# Autodesk Inventor assembly: HalfLeftTest
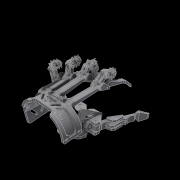
[picture p0: Inventor's stored thumbnail of the model, 180x180]
Saved by Autodesk Inventor 2015 (Build 190159000, 159)
## iProperties
Created: 2014-10-25
Part Number: HalfLeftTest
Document SubType Name: Assembly
Designer: Val
Mass: 54.0122 g
Surface Area: 465.408 cm^2
Volume: 54.0122 cm^3
Density: 1 g/cm^3
Author: Val
## Documents named in this file (31)
- F:\Exo\Models\3D\HandLeft.iam
- F:\Exo\Models\3D\HandShockPlateLeft.ipt
- F:\Exo\Models\3D\VibroKnuckle.ipt
- F:\Exo\Models\3D\KnuckleSide.ipt
- F:\Exo\Models\3D\ThumbShockPlateLeft.ipt
- F:\Exo\Models\3D\ThumbMount.ipt
- F:\Exo\Models\3D\MetacarpusIndex.ipt
- F:\Exo\Models\3D\MetacarpusMiddle.ipt
- F:\Exo\Models\3D\MetacarpusRing.ipt
- F:\Exo\Models\3D\MetacarpusPinky.ipt
- F:\Exo\Models\3D\MetacarpusThumb.ipt
- F:\Exo\Models\3D\ProxPhalangeIndex.ipt
- F:\Exo\Models\3D\ProxPhalangeMiddle.ipt
- F:\Exo\Models\3D\ProxPhalangeRing.ipt
- F:\Exo\Models\3D\ProxPhalangePinky.ipt
- F:\Exo\Models\3D\DistPhalangeIndex.ipt
- F:\Exo\Models\3D\DistPhalangeMiddle.ipt
- F:\Exo\Models\3D\DistPhalangeRing.ipt
- F:\Exo\Models\3D\DistPhalangePinky.ipt
- F:\Exo\Models\3D\DistPhalangeThumb.ipt
- F:\Exo\Models\3D\HandRibLeft.ipt
- F:\Exo\Models\3D\IndexRouter.ipt
- F:\Exo\Models\3D\MiddleRouter.ipt
- F:\Exo\Models\3D\RingRouter.ipt
- F:\Exo\Models\3D\PinkyRouter.ipt
- F:\Exo\Models\3D\ThumbRouter.ipt
- F:\Exo\Models\3D\VibroMount.ipt
- F:\Exo\Models\3D\ChainLink.ipt
- F:\Exo\Models\3D\ChainTooth.ipt
- F:\Exo\Models\3D\ChainGear.ipt
- F:\Exo\Models\3D\ProxPhalangeThumb.ipt
## Components (167 placed, 30 different names)
1. HandShockPlateLeft:1 — Mate:72, Mate:73, Mate:78, Mate:79, Mate:80, Mate:81, Mate:137, Mate:139
2. ThumbShockPlateLeft:1 — Mate:72, Mate:73, Mate:74, Mate:75
3. ThumbMount:1 — Mate:74, Mate:75, Mate:76, Mate:77
4. VibroKnuckle:1 — Mate:82, Mate:83, Mate:94, Mate:95, Mate:410, Mate:411, Mate:413
5. VibroKnuckle:2 — Mate:84, Mate:85, Mate:96, Mate:97, Mate:347, Mate:348, Mate:349, Mate:350
6. VibroKnuckle:3 — Mate:86, Mate:87, Mate:98, Mate:99, Mate:142, Mate:143, Mate:144, Mate:145
7. VibroKnuckle:4 — Mate:88, Mate:89, Mate:286, Mate:287
8. VibroKnuckle:5 — Mate:90, Mate:91, Mate:100, Mate:101, Mate:283, Mate:284, Mate:285
9. KnuckleSide:1 — Mate:102, Mate:104
10. KnuckleSide:2 — Mate:105, Mate:107
11. KnuckleSide:3 — Mate:108, Mate:109, Mate:110
12. KnuckleSide:4 — Mate:111, Mate:112, Mate:113
13. KnuckleSide:5 — Mate:114, Mate:115, Mate:116
14. KnuckleSide:6 — Mate:117, Mate:118, Mate:119
15. KnuckleSide:7 — Mate:120, Mate:121, Mate:122
16. KnuckleSide:8 — Mate:123, Mate:124, Mate:125
17. KnuckleSide:9 — Mate:129, Mate:130, Mate:131
18. KnuckleSide:10 — Mate:126, Mate:127, Mate:128
19. MetacarpusIndex:1 — Mate:78, Mate:82, Mate:83, Mate:108, Mate:110, Mate:111, Mate:113
20. MetacarpusMiddle:2 — Mate:79, Mate:84, Mate:85, Mate:114, Mate:116, Mate:117, Mate:119
21. MetacarpusRing:3 — Mate:80, Mate:86, Mate:87, Mate:120, Mate:122, Mate:123, Mate:125
22. MetacarpusPinky:4 — Mate:81, Mate:90, Mate:91, Mate:126, Mate:128, Mate:129, Mate:131
23. MetacarpusThumb:5 — Mate:76, Mate:77, Mate:88, Mate:89, Mate:102, Mate:104, Mate:105, Mate:107
24. ProxPhalangeIndex:1 — Mate:94, Mate:95, Mate:109, Mate:112, Mate:135
25. ProxPhalangeMiddle:2 — Mate:96, Mate:97, Mate:115, Mate:118, Mate:134
26. ProxPhalangeRing:3 — Mate:98, Mate:99, Mate:121, Mate:124, Mate:133
27. ProxPhalangePinky:4 — Mate:100, Mate:101, Mate:127, Mate:130, Mate:132
28. DistPhalangeIndex:1 — Mate:135
29. DistPhalangeMiddle:1 — Mate:134
30. DistPhalangeRing:1 — Mate:133
31. DistPhalangePinky:1 — Mate:132
32. DistPhalangeThumb:1
33. HandRibLeft:1 — Mate:137, Mate:139
34. IndexRouter:1
35. MiddleRouter:1
36. RingRouter:1
37. PinkyRouter:1
38. ThumbRouter:1
39. VibroMount:1 — Mate:142, Mate:143, Mate:148, Mate:180
40. VibroMount:2 — Mate:144, Mate:145, Mate:148, Mate:179
41. ChainLink:1 — Mate:149, Mate:150, Mate:181
42. ChainTooth:1 — Mate:149, Mate:150, Mate:151, Mate:152, Mate:154, Mate:155, Mate:156, Flush:4, Flush:15
43. ChainLink:2 — Mate:156, Flush:1, Mate:181, Mate:216
44. ChainLink:3 — Mate:154, Mate:155, Flush:1, Mate:178
45. ChainLink:4 — Mate:151, Mate:152, Mate:171
46. ChainLink:7 — Mate:172
47. ChainTooth:2 — Flush:5, Flush:6
48. ChainLink:8 — Mate:173
49. ChainLink:9 — Mate:176
50. ChainLink:10 — Mate:174
51. ChainLink:11 — Mate:175
52. ChainTooth:3 — Flush:7
53. ChainLink:12 — Mate:177
54. ChainLink:13 — Mate:182
55. ChainLink:14 — Mate:182, Mate:222, Mate:223
56. ChainTooth:4 — Mate:171, Flush:4, Flush:5, Mate:172, Mate:173, Mate:178
57. ChainTooth:5 — Flush:6, Mate:174, Flush:7, Mate:175, Mate:176, Mate:177
58. VibroKnuckle:6 — Mate:179, Mate:180, Mate:218, Mate:219, Mate:220, Mate:221
59. ChainTooth:7 — Mate:223
60. ChainLink:21
61. ChainLink:22
62. ChainLink:23
63. ChainTooth:8
64. ChainLink:24
65. ChainLink:25 — Mate:215
66. ChainLink:26 — Mate:214
67. ChainTooth:10
68. ChainTooth:11 — Mate:214, Mate:215, Mate:216, Flush:15
69. ChainGear:1 — Mate:218, Mate:220, Mate:222
70. ChainGear:2 — Mate:219, Mate:221
71. VibroMount:3 — Mate:285
72. VibroMount:4 — Mate:283, Mate:284
73. ChainLink:27 — Flush:36, Flush:37
74. ChainTooth:12
75. ChainLink:28
76. ChainLink:29
77. ChainLink:30 — Flush:28, Flush:29, Flush:37
78. ChainLink:31 — Flush:29, Flush:30
79. ChainTooth:13
80. ChainLink:32
81. ChainLink:33
82. ChainLink:34 — Flush:30, Flush:31
83. ChainLink:35 — Flush:27, Flush:31, Flush:32
84. ChainTooth:14
85. ChainLink:36
86. ChainLink:37
87. ChainLink:38 — Flush:32, Flush:33
88. ChainTooth:15
89. ChainTooth:16
90. VibroKnuckle:7
91. ChainTooth:17
92. ChainLink:39
93. ChainLink:40 — Flush:33, Flush:34
94. ChainLink:41 — Flush:34, Flush:35
95. ChainTooth:18
96. ChainLink:42
97. ChainLink:43
98. ChainLink:44 — Flush:35, Flush:36
99. ChainTooth:19
100. ChainTooth:20
101. ChainGear:3 — Flush:27
102. ChainGear:4 — Flush:28
103. ProxPhalangeThumb:1 — Mate:286, Mate:287
104. VibroMount:5 — Mate:347, Mate:348
105. VibroMount:6 — Mate:349, Mate:350
106. ChainLink:45
107. ChainTooth:21
108. ChainLink:46
109. ChainLink:47
110. ChainLink:48
111. ChainLink:49
112. ChainTooth:22
113. ChainLink:50
114. ChainLink:51
115. ChainLink:52
116. ChainLink:53
117. ChainTooth:23
118. ChainLink:54
119. ChainLink:55
120. ChainLink:56
121. ChainTooth:24
122. ChainTooth:25
123. VibroKnuckle:8
124. ChainTooth:26
125. ChainLink:57
126. ChainLink:58
127. ChainLink:59
128. ChainTooth:27
129. ChainLink:60
130. ChainLink:61
131. ChainLink:62
132. ChainTooth:28
133. ChainTooth:29
134. ChainGear:5
135. ChainGear:6
136. VibroMount:7 — Mate:410, Mate:411, Mate:412
137. VibroMount:8 — Mate:413
138. ChainLink:63
139. ChainTooth:30
140. ChainLink:64
141. ChainLink:65
142. ChainLink:66
143. ChainLink:67
144. ChainTooth:31
145. ChainLink:68
146. ChainLink:69
147. ChainLink:70
148. ChainLink:71
149. ChainTooth:32
150. ChainLink:72
151. ChainLink:73
152. ChainLink:74
153. ChainTooth:33
154. ChainTooth:34
155. VibroKnuckle:9 — Mate:412
156. ChainTooth:35
157. ChainLink:75
158. ChainLink:76
159. ChainLink:77
160. ChainTooth:36
161. ChainLink:78
162. ChainLink:79
163. ChainLink:80
164. ChainTooth:37
165. ChainTooth:38
166. ChainGear:7
167. ChainGear:8
## Relationships (392: Mate 315, Flush 77)
- Mate:72: HandShockPlateLeft:1 ↔ ThumbShockPlateLeft:1
- Mate:73: HandShockPlateLeft:1 ↔ ThumbShockPlateLeft:1
- Mate:74: ThumbShockPlateLeft:1 ↔ ThumbMount:1
- Mate:75: ThumbShockPlateLeft:1 ↔ ThumbMount:1
- Mate:76: ThumbMount:1 ↔ MetacarpusThumb:5
- Mate:77: ThumbMount:1 ↔ MetacarpusThumb:5
- Mate:78: HandShockPlateLeft:1 ↔ MetacarpusIndex:1
- Mate:79: HandShockPlateLeft:1 ↔ MetacarpusMiddle:2
- Mate:80: HandShockPlateLeft:1 ↔ MetacarpusRing:3
- Mate:81: HandShockPlateLeft:1 ↔ MetacarpusPinky:4
- Mate:82: VibroKnuckle:1 ↔ MetacarpusIndex:1
- Mate:83: VibroKnuckle:1 ↔ MetacarpusIndex:1
- Mate:84: VibroKnuckle:2 ↔ MetacarpusMiddle:2
- Mate:85: VibroKnuckle:2 ↔ MetacarpusMiddle:2
- Mate:86: VibroKnuckle:3 ↔ MetacarpusRing:3
- Mate:87: VibroKnuckle:3 ↔ MetacarpusRing:3
- Mate:88: VibroKnuckle:4 ↔ MetacarpusThumb:5
- Mate:89: VibroKnuckle:4 ↔ MetacarpusThumb:5
- Mate:90: VibroKnuckle:5 ↔ MetacarpusPinky:4
- Mate:91: VibroKnuckle:5 ↔ MetacarpusPinky:4
- Mate:94: VibroKnuckle:1 ↔ ProxPhalangeIndex:1
- Mate:95: VibroKnuckle:1 ↔ ProxPhalangeIndex:1
- Mate:96: VibroKnuckle:2 ↔ ProxPhalangeMiddle:2
- Mate:97: VibroKnuckle:2 ↔ ProxPhalangeMiddle:2
- Mate:98: VibroKnuckle:3 ↔ ProxPhalangeRing:3
- Mate:99: VibroKnuckle:3 ↔ ProxPhalangeRing:3
- Mate:100: VibroKnuckle:5 ↔ ProxPhalangePinky:4
- Mate:101: VibroKnuckle:5 ↔ ProxPhalangePinky:4
- Mate:102: KnuckleSide:1 ↔ MetacarpusThumb:5
- Mate:104: KnuckleSide:1 ↔ MetacarpusThumb:5
- Mate:105: KnuckleSide:2 ↔ MetacarpusThumb:5
- Mate:107: KnuckleSide:2 ↔ MetacarpusThumb:5
- Mate:108: KnuckleSide:3 ↔ MetacarpusIndex:1
- Mate:109: KnuckleSide:3 ↔ ProxPhalangeIndex:1
- Mate:110: KnuckleSide:3 ↔ MetacarpusIndex:1
- Mate:111: KnuckleSide:4 ↔ MetacarpusIndex:1
- Mate:112: KnuckleSide:4 ↔ ProxPhalangeIndex:1
- Mate:113: KnuckleSide:4 ↔ MetacarpusIndex:1
- Mate:114: KnuckleSide:5 ↔ MetacarpusMiddle:2
- Mate:115: KnuckleSide:5 ↔ ProxPhalangeMiddle:2
- Mate:116: KnuckleSide:5 ↔ MetacarpusMiddle:2
- Mate:117: KnuckleSide:6 ↔ MetacarpusMiddle:2
- Mate:118: KnuckleSide:6 ↔ ProxPhalangeMiddle:2
- Mate:119: KnuckleSide:6 ↔ MetacarpusMiddle:2
- Mate:120: KnuckleSide:7 ↔ MetacarpusRing:3
- Mate:121: KnuckleSide:7 ↔ ProxPhalangeRing:3
- Mate:122: KnuckleSide:7 ↔ MetacarpusRing:3
- Mate:123: KnuckleSide:8 ↔ MetacarpusRing:3
- Mate:124: KnuckleSide:8 ↔ ProxPhalangeRing:3
- Mate:125: KnuckleSide:8 ↔ MetacarpusRing:3
- Mate:126: KnuckleSide:10 ↔ MetacarpusPinky:4
- Mate:127: KnuckleSide:10 ↔ ProxPhalangePinky:4
- Mate:128: KnuckleSide:10 ↔ MetacarpusPinky:4
- Mate:129: KnuckleSide:9 ↔ MetacarpusPinky:4
- Mate:130: KnuckleSide:9 ↔ ProxPhalangePinky:4
- Mate:131: KnuckleSide:9 ↔ MetacarpusPinky:4
- Mate:132: ProxPhalangePinky:4 ↔ DistPhalangePinky:1
- Mate:133: ProxPhalangeRing:3 ↔ DistPhalangeRing:1
- Mate:134: ProxPhalangeMiddle:2 ↔ DistPhalangeMiddle:1
- Mate:135: ProxPhalangeIndex:1 ↔ DistPhalangeIndex:1
- Mate:137: HandShockPlateLeft:1 ↔ HandRibLeft:1
- Mate:139: HandShockPlateLeft:1 ↔ HandRibLeft:1
- Mate:142: VibroKnuckle:3 ↔ VibroMount:1
- Mate:143: VibroKnuckle:3 ↔ VibroMount:1
- Mate:144: VibroKnuckle:3 ↔ VibroMount:2
- Mate:145: VibroKnuckle:3 ↔ VibroMount:2
- Mate:148: VibroMount:1 ↔ VibroMount:2
- Mate:149: ChainLink:1 ↔ ChainTooth:1
- Mate:150: ChainLink:1 ↔ ChainTooth:1
- Mate:151: ChainTooth:1 ↔ ChainLink:4
- Mate:152: ChainTooth:1 ↔ ChainLink:4
- Mate:154: ChainTooth:1 ↔ ChainLink:3
- Mate:155: ChainTooth:1 ↔ ChainLink:3
- Mate:156: ChainTooth:1 ↔ ChainLink:2
- Flush:1: ChainLink:2 ↔ ChainLink:3
- [Mate]: ChainLink:7 ↔ ChainTooth:2
- [Mate]: ChainLink:7 ↔ ChainTooth:2
- [Mate]: ChainTooth:2 ↔ ChainLink:10
- [Mate]: ChainTooth:2 ↔ ChainLink:10
- [Mate]: ChainTooth:2 ↔ ChainLink:9
- [Mate]: ChainTooth:2 ↔ ChainLink:9
- [Mate]: ChainTooth:2 ↔ ChainLink:8
- [Flush]: ChainLink:8 ↔ ChainLink:9
- [Mate]: ChainLink:11 ↔ ChainTooth:3
- [Mate]: ChainLink:11 ↔ ChainTooth:3
- [Mate]: ChainTooth:3 ↔ ChainLink:14
- [Mate]: ChainTooth:3 ↔ ChainLink:14
- [Mate]: ChainTooth:3 ↔ ChainLink:13
- [Mate]: ChainTooth:3 ↔ ChainLink:13
- [Mate]: ChainTooth:3 ↔ ChainLink:12
- [Flush]: ChainLink:12 ↔ ChainLink:13
- Mate:171: ChainLink:4 ↔ ChainTooth:4
- Flush:4: ChainTooth:1 ↔ ChainTooth:4
- Flush:5: ChainTooth:2 ↔ ChainTooth:4
- Mate:172: ChainLink:7 ↔ ChainTooth:4
- Mate:173: ChainLink:8 ↔ ChainTooth:4
- Flush:6: ChainTooth:2 ↔ ChainTooth:5
- Mate:174: ChainLink:10 ↔ ChainTooth:5
- Flush:7: ChainTooth:3 ↔ ChainTooth:5
- Mate:175: ChainLink:11 ↔ ChainTooth:5
- Mate:176: ChainLink:9 ↔ ChainTooth:5
- Mate:177: ChainLink:12 ↔ ChainTooth:5
- Mate:178: ChainLink:3 ↔ ChainTooth:4
- Mate:179: VibroMount:2 ↔ VibroKnuckle:6
- Mate:180: VibroMount:1 ↔ VibroKnuckle:6
- Mate:181: ChainLink:1 ↔ ChainLink:2
- Mate:182: ChainLink:13 ↔ ChainLink:14
- [Mate]: ChainTooth:7 ↔ ChainLink:22
- [Mate]: ChainTooth:7 ↔ ChainLink:22
- [Mate]: ChainTooth:7 ↔ ChainLink:21
- [Mate]: ChainTooth:7 ↔ ChainLink:21
- [Mate]: ChainLink:23 ↔ ChainTooth:8
- [Mate]: ChainLink:23 ↔ ChainTooth:8
- [Mate]: ChainTooth:8 ↔ ChainLink:26
- [Mate]: ChainTooth:8 ↔ ChainLink:26
- [Mate]: ChainTooth:8 ↔ ChainLink:25
- [Mate]: ChainTooth:8 ↔ ChainLink:25
- [Mate]: ChainTooth:8 ↔ ChainLink:24
- [Flush]: ChainLink:24 ↔ ChainLink:25
- [Flush]: ChainTooth:7 ↔ ChainTooth:10
- [Mate]: ChainLink:22 ↔ ChainTooth:10
- [Flush]: ChainTooth:8 ↔ ChainTooth:10
- [Mate]: ChainLink:23 ↔ ChainTooth:10
- [Mate]: ChainLink:21 ↔ ChainTooth:10
- [Mate]: ChainLink:24 ↔ ChainTooth:10
- [Mate]: ChainLink:25 ↔ ChainLink:26
- Mate:214: ChainLink:26 ↔ ChainTooth:11
- Mate:215: ChainLink:25 ↔ ChainTooth:11
- Mate:216: ChainLink:2 ↔ ChainTooth:11
- Flush:15: ChainTooth:1 ↔ ChainTooth:11
- Mate:218: VibroKnuckle:6 ↔ ChainGear:1
- Mate:219: VibroKnuckle:6 ↔ ChainGear:2
- Mate:220: VibroKnuckle:6 ↔ ChainGear:1
- Mate:221: VibroKnuckle:6 ↔ ChainGear:2
- Mate:222: ChainLink:14 ↔ ChainGear:1
- Mate:223: ChainLink:14 ↔ ChainTooth:7
- [Mate]: VibroMount:3 ↔ VibroMount:4
- [Mate]: ChainLink:27 ↔ ChainTooth:12
- [Mate]: ChainLink:27 ↔ ChainTooth:12
- [Mate]: ChainTooth:12 ↔ ChainLink:30
- [Mate]: ChainTooth:12 ↔ ChainLink:30
- [Mate]: ChainTooth:12 ↔ ChainLink:29
- [Mate]: ChainTooth:12 ↔ ChainLink:29
- [Mate]: ChainTooth:12 ↔ ChainLink:28
- [Flush]: ChainLink:28 ↔ ChainLink:29
- [Mate]: ChainLink:31 ↔ ChainTooth:13
- [Mate]: ChainLink:31 ↔ ChainTooth:13
- [Mate]: ChainTooth:13 ↔ ChainLink:34
- [Mate]: ChainTooth:13 ↔ ChainLink:34
- [Mate]: ChainTooth:13 ↔ ChainLink:33
- [Mate]: ChainTooth:13 ↔ ChainLink:33
- [Mate]: ChainTooth:13 ↔ ChainLink:32
- [Flush]: ChainLink:32 ↔ ChainLink:33
- [Mate]: ChainLink:35 ↔ ChainTooth:14
- [Mate]: ChainLink:35 ↔ ChainTooth:14
- [Mate]: ChainTooth:14 ↔ ChainLink:38
- [Mate]: ChainTooth:14 ↔ ChainLink:38
- [Mate]: ChainTooth:14 ↔ ChainLink:37
- [Mate]: ChainTooth:14 ↔ ChainLink:37
- [Mate]: ChainTooth:14 ↔ ChainLink:36
- [Flush]: ChainLink:36 ↔ ChainLink:37
- [Mate]: ChainLink:30 ↔ ChainTooth:15
- [Flush]: ChainTooth:12 ↔ ChainTooth:15
- [Flush]: ChainTooth:13 ↔ ChainTooth:15
- [Mate]: ChainLink:31 ↔ ChainTooth:15
- [Mate]: ChainLink:32 ↔ ChainTooth:15
- [Flush]: ChainTooth:13 ↔ ChainTooth:16
- [Mate]: ChainLink:34 ↔ ChainTooth:16
- [Flush]: ChainTooth:14 ↔ ChainTooth:16
- [Mate]: ChainLink:35 ↔ ChainTooth:16
- [Mate]: ChainLink:33 ↔ ChainTooth:16
- [Mate]: ChainLink:36 ↔ ChainTooth:16
- [Mate]: ChainLink:29 ↔ ChainTooth:15
- [Mate]: VibroMount:4 ↔ VibroKnuckle:7
- [Mate]: VibroMount:3 ↔ VibroKnuckle:7
- [Mate]: ChainLink:27 ↔ ChainLink:28
- [Mate]: ChainLink:37 ↔ ChainLink:38
- [Mate]: ChainTooth:17 ↔ ChainLink:40
- [Mate]: ChainTooth:17 ↔ ChainLink:40
- [Mate]: ChainTooth:17 ↔ ChainLink:39
- [Mate]: ChainTooth:17 ↔ ChainLink:39
- [Mate]: ChainLink:41 ↔ ChainTooth:18
- [Mate]: ChainLink:41 ↔ ChainTooth:18
- [Mate]: ChainTooth:18 ↔ ChainLink:44
- [Mate]: ChainTooth:18 ↔ ChainLink:44
- [Mate]: ChainTooth:18 ↔ ChainLink:43
- [Mate]: ChainTooth:18 ↔ ChainLink:43
- [Mate]: ChainTooth:18 ↔ ChainLink:42
- [Flush]: ChainLink:42 ↔ ChainLink:43
- [Flush]: ChainTooth:17 ↔ ChainTooth:19
- [Mate]: ChainLink:40 ↔ ChainTooth:19
- [Flush]: ChainTooth:18 ↔ ChainTooth:19
- [Mate]: ChainLink:41 ↔ ChainTooth:19
- [Mate]: ChainLink:39 ↔ ChainTooth:19
- [Mate]: ChainLink:42 ↔ ChainTooth:19
- [Mate]: ChainLink:43 ↔ ChainLink:44
- [Mate]: ChainLink:44 ↔ ChainTooth:20
- [Mate]: ChainLink:43 ↔ ChainTooth:20
- [Mate]: ChainLink:28 ↔ ChainTooth:20
- [Flush]: ChainTooth:12 ↔ ChainTooth:20
- [Mate]: VibroKnuckle:7 ↔ ChainGear:3
- [Mate]: VibroKnuckle:7 ↔ ChainGear:4
- [Mate]: VibroKnuckle:7 ↔ ChainGear:3
- [Mate]: VibroKnuckle:7 ↔ ChainGear:4
- [Mate]: ChainLink:38 ↔ ChainGear:3
- [Mate]: ChainLink:38 ↔ ChainTooth:17
- Flush:27: ChainLink:35 ↔ ChainGear:3
- Flush:28: ChainLink:30 ↔ ChainGear:4
- Flush:29: ChainLink:30 ↔ ChainLink:31
- Flush:30: ChainLink:31 ↔ ChainLink:34
- Flush:31: ChainLink:34 ↔ ChainLink:35
- Flush:32: ChainLink:35 ↔ ChainLink:38
- Flush:33: ChainLink:38 ↔ ChainLink:40
- Flush:34: ChainLink:40 ↔ ChainLink:41
- Flush:35: ChainLink:41 ↔ ChainLink:44
- Flush:36: ChainLink:27 ↔ ChainLink:44
- Flush:37: ChainLink:27 ↔ ChainLink:30
- Mate:283: VibroKnuckle:5 ↔ VibroMount:4
- Mate:284: VibroKnuckle:5 ↔ VibroMount:4
- Mate:285: VibroKnuckle:5 ↔ VibroMount:3
- Mate:286: VibroKnuckle:4 ↔ ProxPhalangeThumb:1
- Mate:287: VibroKnuckle:4 ↔ ProxPhalangeThumb:1
- [Mate]: VibroMount:5 ↔ VibroMount:6
- [Mate]: ChainLink:45 ↔ ChainTooth:21
- [Mate]: ChainLink:45 ↔ ChainTooth:21
- [Mate]: ChainTooth:21 ↔ ChainLink:48
- [Mate]: ChainTooth:21 ↔ ChainLink:48
- [Mate]: ChainTooth:21 ↔ ChainLink:47
- [Mate]: ChainTooth:21 ↔ ChainLink:47
- [Mate]: ChainTooth:21 ↔ ChainLink:46
- [Flush]: ChainLink:46 ↔ ChainLink:47
- [Mate]: ChainLink:49 ↔ ChainTooth:22
- [Mate]: ChainLink:49 ↔ ChainTooth:22
- [Mate]: ChainTooth:22 ↔ ChainLink:52
- [Mate]: ChainTooth:22 ↔ ChainLink:52
- [Mate]: ChainTooth:22 ↔ ChainLink:51
- [Mate]: ChainTooth:22 ↔ ChainLink:51
- [Mate]: ChainTooth:22 ↔ ChainLink:50
- [Flush]: ChainLink:50 ↔ ChainLink:51
- [Mate]: ChainLink:53 ↔ ChainTooth:23
- [Mate]: ChainLink:53 ↔ ChainTooth:23
- [Mate]: ChainTooth:23 ↔ ChainLink:56
- [Mate]: ChainTooth:23 ↔ ChainLink:56
- [Mate]: ChainTooth:23 ↔ ChainLink:55
- [Mate]: ChainTooth:23 ↔ ChainLink:55
- [Mate]: ChainTooth:23 ↔ ChainLink:54
- [Flush]: ChainLink:54 ↔ ChainLink:55
- [Mate]: ChainLink:48 ↔ ChainTooth:24
- [Flush]: ChainTooth:21 ↔ ChainTooth:24
- [Flush]: ChainTooth:22 ↔ ChainTooth:24
- [Mate]: ChainLink:49 ↔ ChainTooth:24
- [Mate]: ChainLink:50 ↔ ChainTooth:24
- [Flush]: ChainTooth:22 ↔ ChainTooth:25
- [Mate]: ChainLink:52 ↔ ChainTooth:25
- [Flush]: ChainTooth:23 ↔ ChainTooth:25
- [Mate]: ChainLink:53 ↔ ChainTooth:25
- [Mate]: ChainLink:51 ↔ ChainTooth:25
- [Mate]: ChainLink:54 ↔ ChainTooth:25
- [Mate]: ChainLink:47 ↔ ChainTooth:24
- [Mate]: VibroMount:6 ↔ VibroKnuckle:8
- [Mate]: VibroMount:5 ↔ VibroKnuckle:8
- [Mate]: ChainLink:45 ↔ ChainLink:46
- [Mate]: ChainLink:55 ↔ ChainLink:56
- [Mate]: ChainTooth:26 ↔ ChainLink:58
- [Mate]: ChainTooth:26 ↔ ChainLink:58
- [Mate]: ChainTooth:26 ↔ ChainLink:57
- [Mate]: ChainTooth:26 ↔ ChainLink:57
- [Mate]: ChainLink:59 ↔ ChainTooth:27
- [Mate]: ChainLink:59 ↔ ChainTooth:27
- [Mate]: ChainTooth:27 ↔ ChainLink:62
- [Mate]: ChainTooth:27 ↔ ChainLink:62
- [Mate]: ChainTooth:27 ↔ ChainLink:61
- [Mate]: ChainTooth:27 ↔ ChainLink:61
- [Mate]: ChainTooth:27 ↔ ChainLink:60
- [Flush]: ChainLink:60 ↔ ChainLink:61
- [Flush]: ChainTooth:26 ↔ ChainTooth:28
- [Mate]: ChainLink:58 ↔ ChainTooth:28
- [Flush]: ChainTooth:27 ↔ ChainTooth:28
- [Mate]: ChainLink:59 ↔ ChainTooth:28
- [Mate]: ChainLink:57 ↔ ChainTooth:28
- [Mate]: ChainLink:60 ↔ ChainTooth:28
- [Mate]: ChainLink:61 ↔ ChainLink:62
- [Mate]: ChainLink:62 ↔ ChainTooth:29
- [Mate]: ChainLink:61 ↔ ChainTooth:29
- [Mate]: ChainLink:46 ↔ ChainTooth:29
- [Flush]: ChainTooth:21 ↔ ChainTooth:29
- [Mate]: VibroKnuckle:8 ↔ ChainGear:5
- [Mate]: VibroKnuckle:8 ↔ ChainGear:6
- [Mate]: VibroKnuckle:8 ↔ ChainGear:5
- [Mate]: VibroKnuckle:8 ↔ ChainGear:6
- [Mate]: ChainLink:56 ↔ ChainGear:5
- [Mate]: ChainLink:56 ↔ ChainTooth:26
- [Flush]: ChainLink:53 ↔ ChainGear:5
- [Flush]: ChainLink:48 ↔ ChainGear:6
- [Flush]: ChainLink:48 ↔ ChainLink:49
- [Flush]: ChainLink:49 ↔ ChainLink:52
- [Flush]: ChainLink:52 ↔ ChainLink:53
- [Flush]: ChainLink:53 ↔ ChainLink:56
- [Flush]: ChainLink:56 ↔ ChainLink:58
- [Flush]: ChainLink:58 ↔ ChainLink:59
- [Flush]: ChainLink:59 ↔ ChainLink:62
- [Flush]: ChainLink:45 ↔ ChainLink:62
- [Flush]: ChainLink:45 ↔ ChainLink:48
- Mate:347: VibroKnuckle:2 ↔ VibroMount:5
- Mate:348: VibroKnuckle:2 ↔ VibroMount:5
- Mate:349: VibroKnuckle:2 ↔ VibroMount:6
- Mate:350: VibroKnuckle:2 ↔ VibroMount:6
- [Mate]: VibroMount:7 ↔ VibroMount:8
- [Mate]: ChainLink:63 ↔ ChainTooth:30
- [Mate]: ChainLink:63 ↔ ChainTooth:30
- [Mate]: ChainTooth:30 ↔ ChainLink:66
- [Mate]: ChainTooth:30 ↔ ChainLink:66
- [Mate]: ChainTooth:30 ↔ ChainLink:65
- [Mate]: ChainTooth:30 ↔ ChainLink:65
- [Mate]: ChainTooth:30 ↔ ChainLink:64
- [Flush]: ChainLink:64 ↔ ChainLink:65
- [Mate]: ChainLink:67 ↔ ChainTooth:31
- [Mate]: ChainLink:67 ↔ ChainTooth:31
- [Mate]: ChainTooth:31 ↔ ChainLink:70
- [Mate]: ChainTooth:31 ↔ ChainLink:70
- [Mate]: ChainTooth:31 ↔ ChainLink:69
- [Mate]: ChainTooth:31 ↔ ChainLink:69
- [Mate]: ChainTooth:31 ↔ ChainLink:68
- [Flush]: ChainLink:68 ↔ ChainLink:69
- [Mate]: ChainLink:71 ↔ ChainTooth:32
- [Mate]: ChainLink:71 ↔ ChainTooth:32
- [Mate]: ChainTooth:32 ↔ ChainLink:74
- [Mate]: ChainTooth:32 ↔ ChainLink:74
- [Mate]: ChainTooth:32 ↔ ChainLink:73
- [Mate]: ChainTooth:32 ↔ ChainLink:73
- [Mate]: ChainTooth:32 ↔ ChainLink:72
- [Flush]: ChainLink:72 ↔ ChainLink:73
- [Mate]: ChainLink:66 ↔ ChainTooth:33
- [Flush]: ChainTooth:30 ↔ ChainTooth:33
- [Flush]: ChainTooth:31 ↔ ChainTooth:33
- [Mate]: ChainLink:67 ↔ ChainTooth:33
- [Mate]: ChainLink:68 ↔ ChainTooth:33
- [Flush]: ChainTooth:31 ↔ ChainTooth:34
- [Mate]: ChainLink:70 ↔ ChainTooth:34
- [Flush]: ChainTooth:32 ↔ ChainTooth:34
- [Mate]: ChainLink:71 ↔ ChainTooth:34
- [Mate]: ChainLink:69 ↔ ChainTooth:34
- [Mate]: ChainLink:72 ↔ ChainTooth:34
- [Mate]: ChainLink:65 ↔ ChainTooth:33
- [Mate]: VibroMount:8 ↔ VibroKnuckle:9
- [Mate]: VibroMount:7 ↔ VibroKnuckle:9
- [Mate]: ChainLink:63 ↔ ChainLink:64
- [Mate]: ChainLink:73 ↔ ChainLink:74
- [Mate]: ChainTooth:35 ↔ ChainLink:76
- [Mate]: ChainTooth:35 ↔ ChainLink:76
- [Mate]: ChainTooth:35 ↔ ChainLink:75
- [Mate]: ChainTooth:35 ↔ ChainLink:75
- [Mate]: ChainLink:77 ↔ ChainTooth:36
- [Mate]: ChainLink:77 ↔ ChainTooth:36
- [Mate]: ChainTooth:36 ↔ ChainLink:80
- [Mate]: ChainTooth:36 ↔ ChainLink:80
- [Mate]: ChainTooth:36 ↔ ChainLink:79
- [Mate]: ChainTooth:36 ↔ ChainLink:79
- [Mate]: ChainTooth:36 ↔ ChainLink:78
- [Flush]: ChainLink:78 ↔ ChainLink:79
- [Flush]: ChainTooth:35 ↔ ChainTooth:37
- [Mate]: ChainLink:76 ↔ ChainTooth:37
- [Flush]: ChainTooth:36 ↔ ChainTooth:37
- [Mate]: ChainLink:77 ↔ ChainTooth:37
- [Mate]: ChainLink:75 ↔ ChainTooth:37
- [Mate]: ChainLink:78 ↔ ChainTooth:37
- [Mate]: ChainLink:79 ↔ ChainLink:80
- [Mate]: ChainLink:80 ↔ ChainTooth:38
- [Mate]: ChainLink:79 ↔ ChainTooth:38
- [Mate]: ChainLink:64 ↔ ChainTooth:38
- [Flush]: ChainTooth:30 ↔ ChainTooth:38
- [Mate]: VibroKnuckle:9 ↔ ChainGear:7
- [Mate]: VibroKnuckle:9 ↔ ChainGear:8
- [Mate]: VibroKnuckle:9 ↔ ChainGear:7
- [Mate]: VibroKnuckle:9 ↔ ChainGear:8
- [Mate]: ChainLink:74 ↔ ChainGear:7
- [Mate]: ChainLink:74 ↔ ChainTooth:35
- [Flush]: ChainLink:71 ↔ ChainGear:7
- [Flush]: ChainLink:66 ↔ ChainGear:8
- [Flush]: ChainLink:66 ↔ ChainLink:67
- [Flush]: ChainLink:67 ↔ ChainLink:70
- [Flush]: ChainLink:70 ↔ ChainLink:71
- [Flush]: ChainLink:71 ↔ ChainLink:74
- [Flush]: ChainLink:74 ↔ ChainLink:76
- [Flush]: ChainLink:76 ↔ ChainLink:77
- [Flush]: ChainLink:77 ↔ ChainLink:80
- [Flush]: ChainLink:63 ↔ ChainLink:80
- [Flush]: ChainLink:63 ↔ ChainLink:66
- Mate:410: VibroKnuckle:1 ↔ VibroMount:7
- Mate:411: VibroKnuckle:1 ↔ VibroMount:7
- Mate:412: VibroMount:7 ↔ VibroKnuckle:9
- Mate:413: VibroKnuckle:1 ↔ VibroMount:8
## Named parameters: d206_d196 = 0 mm, d207_d197 = 0 mm, d208_d198 = 0 mm, d209_d199 = 0 mm, d210_d201 = 0 mm, d211_d202 = 0 mm, d212_d204 = 0 mm, d213_d205 = 0 mm, d214_d196 = 0 mm, d215_d197 = 0 mm, d216_d198 = 0 mm, d217_d199 = 0 mm, d218_d201 = 0 mm, d219_d202 = 0 mm, d220_d204 = 0 mm, d221_d205 = 0 mm, d240_d228 = 0 mm, d241_d229 = 0 mm, d242_d230 = 0 mm, d243_d231 = 0 mm, d244_d232 = 0 mm, d247_d239 = 0 mm, d257_d208_d198 = 0 mm, d258_d209_d199 = 0 mm, d259_d210_d201 = 0 mm, d260_d211_d202 = 0 mm, d263_d214_d196 = 0 mm, d264_d215_d197 = 0 mm, d265_d216_d198 = 0 mm, d266_d217_d199 = 0 mm, d267_d218_d201 = 0 mm, d268_d219_d202 = 0 mm, d269_d220_d204 = 0 mm, d270_d221_d205 = 0 mm, d276_d227 = 0 mm, d290_d266_d217_d199 = 0 mm, d291_d267_d218_d201 = 0 mm, d292_d268_d219_d202 = 0 mm, d293_d269_d220_d204 = 0 mm, d294_d270_d221_d205 = 0 mm, d295_d276_d227 = 0 mm, d296_d278 = 0 mm, d297_d279 = 0 mm, d298_d280 = 0 mm, d299_d281 = 0 mm, d300_d283 = 0 mm, d301_d228 = 0 mm, d302_d229 = 0 mm, d303_d230 = 0 mm, d304_d231 = 0 mm, d305_d232 = 0 mm, d306_d233 = 0 mm, d307_d236 = 0 mm, d308_d237 = 0 mm, d309_d238 = 0 mm, d310_d239 = 0 mm, d311_d240_d228 = 0 mm, d312_d241_d229 = 0 mm, d313_d242_d230 = 0 mm, d314_d243_d231 = 0 mm, d315_d244_d232 = 0 mm, d316_d247_d239 = 0 mm, d317_d257_d208_d198 = 0 mm, d318_d258_d209_d199 = 0 mm, d319_d259_d210_d201 = 0 mm, d320_d260_d211_d202 = 0 mm, d321_d263_d214_d196 = 0 mm, d322_d264_d215_d197 = 0 mm, d323_d265_d216_d198 = 0 mm, d324_d285 = 0 mm, d325_d286 = 0 mm, d326_d287 = 0 mm, d327_d288 = 0 mm, d328_d289 = 0 mm, d329_d197 = 0 mm, d330_d198 = 0 mm, d331_d199 = 0 mm, d332_d201 = 0 mm, d333_d202 = 0 mm, d334_d204 = 0 mm, d335_d205 = 0 mm, d336_d206_d196 = 0 mm, d337_d207_d197 = 0 mm, d338_d208_d198 = 0 mm, d339_d209_d199 = 0 mm, d340_d210_d201 = 0 mm, d341_d211_d202 = 0 mm, d342_d212_d204 = 0 mm, d343_d213_d205 = 0 mm, d344_d214_d196 = 0 mm, d345_d215_d197 = 0 mm, d346_d216_d198 = 0 mm, d347_d217_d199 = 0 mm, d348_d218_d201 = 0 mm, d349_d219_d202 = 0 mm, d350_d220_d204 = 0 mm, d351_d221_d205 = 0 mm, d352_d222 = 0 mm, d353_d223 = 0 mm, d354_d224 = 0 mm, d355_d225 = 0 mm, d356_d226 = 0 mm, d357_d227 = 0 mm, d358_d195 = 0 mm, d359_d196 = 0 mm, d376_d348_d218_d201 = 0 mm, d377_d349_d219_d202 = 0 mm, d378_d350_d220_d204 = 0 mm, d379_d351_d221_d205 = 0 mm, d380_d352_d222 = 0 mm, d381_d353_d223 = 0 mm, d382_d354_d224 = 0 mm, d383_d355_d225 = 0 mm, d384_d356_d226 = 0 mm, d385_d357_d227 = 0 mm, d386_d358_d195 = 0 mm, d387_d359_d196 = 0 mm, d388_d360 = 0 mm, d389_d290_d266_d217_d199 = 0 mm, d390_d291_d267_d218_d201 = 0 mm, d391_d292_d268_d219_d202 = 0 mm, d392_d293_d269_d220_d204 = 0 mm, d393_d294_d270_d221_d205 = 0 mm, d394_d295_d276_d227 = 0 mm, d395_d296_d278 = 0 mm, d396_d297_d279 = 0 mm, d397_d298_d280 = 0 mm, d398_d299_d281 = 0 mm, d399_d300_d283 = 0 mm, d400_d301_d228 = 0 mm, d401_d302_d229 = 0 mm, d402_d303_d230 = 0 mm, d403_d304_d231 = 0 mm, d404_d305_d232 = 0 mm, d405_d306_d233 = 0 mm, d406_d307_d236 = 0 mm, d407_d308_d237 = 0 mm, d408_d309_d238 = 0 mm, d409_d310_d239 = 0 mm, d410_d311_d240_d228 = 0 mm, d411_d312_d241_d229 = 0 mm, d412_d313_d242_d230 = 0 mm, d413_d314_d243_d231 = 0 mm, d414_d315_d244_d232 = 0 mm, d415_d316_d247_d239 = 0 mm, d416_d317_d257_d208_d198 = 0 mm, d417_d318_d258_d209_d199 = 0 mm, d418_d319_d259_d210_d201 = 0 mm, d419_d320_d260_d211_d202 = 0 mm, d420_d321_d263_d214_d196 = 0 mm, d421_d322_d264_d215_d197 = 0 mm, d422_d323_d265_d216_d198 = 0 mm, d423_d324_d285 = 0 mm, d424_d325_d286 = 0 mm, d425_d326_d287 = 0 mm, d426_d327_d288 = 0 mm, d427_d328_d289 = 0 mm, d428_d329_d197 = 0 mm, d429_d330_d198 = 0 mm, d430_d331_d199 = 0 mm, d431_d332_d201 = 0 mm, d432_d333_d202 = 0 mm, d433_d334_d204 = 0 mm, d434_d335_d205 = 0 mm, d435_d336_d206_d196 = 0 mm, d436_d337_d207_d197 = 0 mm, d437_d338_d208_d198 = 0 mm, d438_d339_d209_d199 = 0 mm, d439_d340_d210_d201 = 0 mm, d440_d341_d211_d202 = 0 mm, d441_d342_d212_d204 = 0 mm, d442_d343_d213_d205 = 0 mm, d443_d344_d214_d196 = 0 mm, d444_d345_d215_d197 = 0 mm, d445_d346_d216_d198 = 0 mm, d446_d347_d217_d199 = 0 mm, d447_d361 = 0 mm, d448_d362 = 0 mm, d449_d363 = 0 mm, d450_d364 = 0 mm, d451_d365 = 0 mm, d452_d366 = 0 mm, d453_d367 = 0 mm, d454_d368 = 0 mm, d455_d369 = 0 mm, d456_d370 = 0 mm, d461_d348_d218_d201 = 0 mm, d462_d349_d219_d202 = 0 mm, d463_d350_d220_d204 = 0 mm, d464_d351_d221_d205 = 0 mm, d465_d352_d222 = 0 mm, d466_d353_d223 = 0 mm, d467_d354_d224 = 0 mm, d468_d355_d225 = 0 mm, d469_d356_d226 = 0 mm, d470_d357_d227 = 0 mm, d471_d358_d195 = 0 mm, d472_d359_d196 = 0 mm, d473_d360 = 0 mm, d474_d290_d266_d217_d199 = 0 mm, d475_d291_d267_d218_d201 = 0 mm, d476_d292_d268_d219_d202 = 0 mm, d477_d293_d269_d220_d204 = 0 mm, d478_d294_d270_d221_d205 = 0 mm, d479_d295_d276_d227 = 0 mm, d480_d296_d278 = 0 mm, d481_d297_d279 = 0 mm, d482_d298_d280 = 0 mm, d483_d299_d281 = 0 mm, d484_d300_d283 = 0 mm, d485_d301_d228 = 0 mm, d486_d302_d229 = 0 mm, d487_d303_d230 = 0 mm, d488_d304_d231 = 0 mm, d489_d305_d232 = 0 mm, d490_d306_d233 = 0 mm, d491_d307_d236 = 0 mm, d492_d308_d237 = 0 mm, d493_d309_d238 = 0 mm, d494_d310_d239 = 0 mm, d495_d311_d240_d228 = 0 mm, d496_d312_d241_d229 = 0 mm, d497_d313_d242_d230 = 0 mm, d498_d314_d243_d231 = 0 mm, d499_d315_d244_d232 = 0 mm, d500_d316_d247_d239 = 0 mm, d501_d317_d257_d208_d198 = 0 mm, d502_d318_d258_d209_d199 = 0 mm, d503_d319_d259_d210_d201 = 0 mm, d504_d320_d260_d211_d202 = 0 mm, d505_d321_d263_d214_d196 = 0 mm, d506_d322_d264_d215_d197 = 0 mm, d507_d323_d265_d216_d198 = 0 mm, d508_d324_d285 = 0 mm, d509_d325_d286 = 0 mm, d510_d326_d287 = 0 mm, d511_d327_d288 = 0 mm, d512_d328_d289 = 0 mm, d513_d329_d197 = 0 mm, d514_d330_d198 = 0 mm, d515_d331_d199 = 0 mm, d516_d332_d201 = 0 mm, d517_d333_d202 = 0 mm, d518_d334_d204 = 0 mm, d519_d335_d205 = 0 mm, d520_d336_d206_d196 = 0 mm, d521_d337_d207_d197 = 0 mm, d522_d338_d208_d198 = 0 mm, d523_d339_d209_d199 = 0 mm, d524_d340_d210_d201 = 0 mm, d525_d341_d211_d202 = 0 mm, d526_d342_d212_d204 = 0 mm, d527_d343_d213_d205 = 0 mm, d528_d344_d214_d196 = 0 mm, d529_d345_d215_d197 = 0 mm, d530_d346_d216_d198 = 0 mm, d531_d347_d217_d199 = 0 mm, d532_d361 = 0 mm, d533_d362 = 0 mm, d534_d363 = 0 mm, d535_d364 = 0 mm, d536_d365 = 0 mm, d537_d366 = 0 mm, d538_d367 = 0 mm, d539_d368 = 0 mm, d540_d369 = 0 mm, d541_d370 = 0 mm
